# Autodesk Inventor assembly: Roll_Fixation_Set
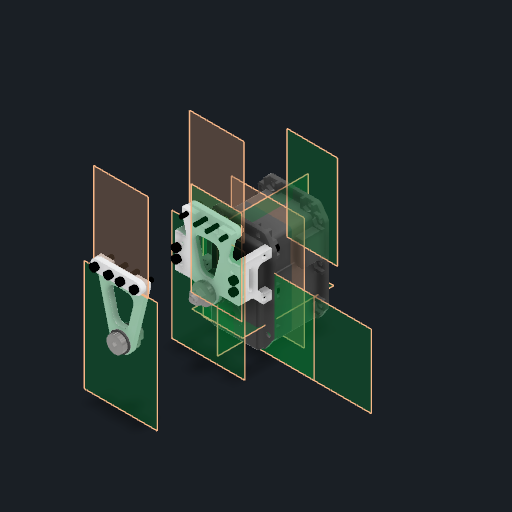
[picture p0: Inventor's stored thumbnail of the model, 512x512]
Saved by Autodesk Inventor 2024.3 (Build 283343000, 343)
## iProperties
Created: 2024-02-15
Part Number: Roll_Fixation_Set
Document SubType Name: Assembly
Designer: ASUS
Author: ASUS
## Documents named in this file (11)
- C:\Users\ASUS\Desktop\Anti_Backlash_Structure_OP\v3_Frame\Roll_Fixation_Set.iam
- C:\Users\ASUS\Desktop\Anti_Backlash_Structure_OP\v3_Frame\Roll_Fixation_Frame.ipt
- C:\Users\ASUS\Desktop\Anti_Backlash_Structure_OP\v3_Frame\Roll_Fixation_Frame_Back.ipt
- C:\Users\ASUS\Desktop\Anti_Backlash_Structure_OP\v3_Frame\hip joint fix washer.ipt
- C:\Users\ASUS\Desktop\Anti_Backlash_Structure_OP\MISUMI\hip_joint_fix_washer_10mm_Set.iam
- C:\Users\ASUS\Desktop\Anti_Backlash_Structure_OP\v3_Frame\Front_Frame_Fixer_v2.iam
- C:\Users\ASUS\Desktop\Anti_Backlash_Structure_OP\v3_Frame\Rear_Frame_Fixer.iam
- C:\Users\ASUS\Desktop\Anti_Backlash_Structure_OP\v3_Frame\Roll_Fixation_Frameto64.ipt
- C:\Users\ASUS\Desktop\Anti_Backlash_Structure_OP\MISUMI\CSH-ST-M2_5-6_203.ipt
- C:\Users\ASUS\Desktop\Anti_Backlash_Structure_OP\ROBOTIS(Inventor 2024 ver.)\DXL\MX-64T.ipt
- C:\Users\ASUS\Desktop\Anti_Backlash_Structure_OP\MISUMI\DBSY4-5-8.ipt
## Components (20 placed, 10 different names)
1. Roll_Fixation_Frame:1 — 메이트:9, 삽입:23
2. Roll_Fixation_Frame_Back:1 — 메이트:9, 삽입:9, 삽입:10, 메이트:12, 메이트:13, 삽입:11, 삽입:12, 삽입:13, 삽입:14, 삽입:25
3. hip joint fix washer:1
4. hip joint fix washer:2
5. hip_joint_fix_washer_10mm_Set:1 [sub-assembly] — 메이트:10, 메이트:11
6. hip_joint_fix_washer_10mm_Set:2 [sub-assembly] — 메이트:10, 메이트:11
7. Front_Frame_Fixer_v2:1 [sub-assembly] — 각도:2, 삽입:22, 삽입:23
8. Rear_Frame_Fixer:1 [sub-assembly] — 각도:1, 각도:2, 삽입:25
9. Roll_Fixation_Frameto64:1 — 삽입:10, 메이트:13, 삽입:16, 삽입:17, 삽입:19, 삽입:20
10. Roll_Fixation_Frameto64:2 — 삽입:9, 메이트:12, 각도:1, 삽입:15, 삽입:18
11. CSH-ST-M2_5-6_203:1 — 삽입:12
12. CSH-ST-M2_5-6_203:2 — 삽입:11
13. CSH-ST-M2_5-6_203:3 — 삽입:13
14. CSH-ST-M2_5-6_203:4 — 삽입:14
15. CSH-ST-M2_5-6_203:5 — 삽입:17
16. CSH-ST-M2_5-6_203:6 — 삽입:16
17. CSH-ST-M2_5-6_203:7 — 삽입:15
18. CSH-ST-M2_5-6_203:8 — 삽입:18
19. MX-64T:1 — 삽입:19, 삽입:20
20. DBSY4-5-8:1 — 삽입:22
## Relationships (34: Insert 20, Mate 12, Angle 2)
- [Mate]: Roll_Fixation_Frame:1 ↔ Roll_Fixation_Frame_Back:1
- [Insert]: Roll_Fixation_Frame:1 ↔ hip joint fix washer:1
- [Insert]: Roll_Fixation_Frame:1 ↔ hip joint fix washer:1
- [Insert]: Roll_Fixation_Frame_Back:1 ↔ hip joint fix washer:2
- [Mate]: Roll_Fixation_Frame_Back:1 ↔ hip joint fix washer:2
- [Mate]: Roll_Fixation_Frame_Back:1 ↔ hip joint fix washer:1
- [Mate]: Roll_Fixation_Frame_Back:1 ↔ hip joint fix washer:1
- [Mate]: Roll_Fixation_Frame:1 ↔ hip joint fix washer:1
- [Insert]: hip joint fix washer:1 ↔ hip_joint_fix_washer_10mm_Set:1
- [Mate]: hip joint fix washer:1 ↔ hip_joint_fix_washer_10mm_Set:1
- [Insert]: hip joint fix washer:2 ↔ hip_joint_fix_washer_10mm_Set:2
- [Mate]: hip joint fix washer:2 ↔ hip_joint_fix_washer_10mm_Set:2
- 메이트:9 [Mate] (49 mm): Roll_Fixation_Frame:1 ↔ Roll_Fixation_Frame_Back:1
- 메이트:10 [Mate]: hip_joint_fix_washer_10mm_Set:1 ↔ hip_joint_fix_washer_10mm_Set:2
- 메이트:11 [Mate]: hip_joint_fix_washer_10mm_Set:1 ↔ hip_joint_fix_washer_10mm_Set:2
- 삽입:9 [Insert]: Roll_Fixation_Frame_Back:1 ↔ Roll_Fixation_Frameto64:2
- 삽입:10 [Insert]: Roll_Fixation_Frame_Back:1 ↔ Roll_Fixation_Frameto64:1
- 메이트:12 [Mate]: Roll_Fixation_Frame_Back:1 ↔ Roll_Fixation_Frameto64:2
- 메이트:13 [Mate]: Roll_Fixation_Frame_Back:1 ↔ Roll_Fixation_Frameto64:1
- 삽입:11 [Insert]: Roll_Fixation_Frame_Back:1 ↔ CSH-ST-M2_5-6_203:2
- 삽입:12 [Insert]: Roll_Fixation_Frame_Back:1 ↔ CSH-ST-M2_5-6_203:1
- 삽입:13 [Insert]: Roll_Fixation_Frame_Back:1 ↔ CSH-ST-M2_5-6_203:3
- 삽입:14 [Insert]: Roll_Fixation_Frame_Back:1 ↔ CSH-ST-M2_5-6_203:4
- 각도:1 [Angle] (0 deg): Rear_Frame_Fixer:1 ↔ Roll_Fixation_Frameto64:2
- 각도:2 [Angle] (0 deg): Front_Frame_Fixer_v2:1 ↔ Rear_Frame_Fixer:1
- 삽입:15 [Insert] (2.5 mm): Roll_Fixation_Frameto64:2 ↔ CSH-ST-M2_5-6_203:7
- 삽입:16 [Insert] (2.5 mm): Roll_Fixation_Frameto64:1 ↔ CSH-ST-M2_5-6_203:6
- 삽입:17 [Insert] (2.5 mm): Roll_Fixation_Frameto64:1 ↔ CSH-ST-M2_5-6_203:5
- 삽입:18 [Insert] (2.5 mm): Roll_Fixation_Frameto64:2 ↔ CSH-ST-M2_5-6_203:8
- 삽입:19 [Insert]: Roll_Fixation_Frameto64:1 ↔ MX-64T:1
- 삽입:20 [Insert]: Roll_Fixation_Frameto64:1 ↔ MX-64T:1
- 삽입:22 [Insert]: Front_Frame_Fixer_v2:1 ↔ DBSY4-5-8:1
- 삽입:23 [Insert]: Roll_Fixation_Frame:1 ↔ Front_Frame_Fixer_v2:1
- 삽입:25 [Insert]: Roll_Fixation_Frame_Back:1 ↔ Rear_Frame_Fixer:1
